# Autodesk Inventor assembly: Air Filter Bracket
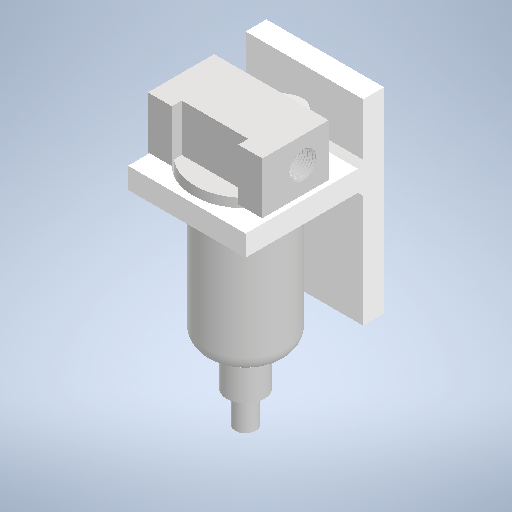
[picture p0: Inventor's stored thumbnail of the model, 512x512]
Saved by Autodesk Inventor 2025 (Build 290162000, 162)
## iProperties
Created: 2025-08-21
Part Number: Air Filter Bracket
Document SubType Name: Assembly
Designer: Caleb Fangmeier
Author: Caleb Fangmeier
## Documents named in this file (3)
- C:\Users\cfang\Desktop\nebraska-silicon-lab\Hardware\General Gantry\Air Filter Bracket\Air Filter Bracket.iam
- C:\Users\cfang\Desktop\nebraska-silicon-lab\Hardware\General Gantry\Air Filter Bracket\4274K91_Compressed Air Filter for Particle Removal\4274K91_Compressed Air Filter for Particle Removal.ipt
- C:\Users\cfang\Desktop\nebraska-silicon-lab\Hardware\General Gantry\Air Filter Bracket\Air Filter Bracket.ipt
## Components (2 placed, 2 different names)
1. 4274K91_Compressed Air Filter for Particle Removal:1 — Insert:1
2. Air Filter Bracket:1 — Insert:1
## Relationships (1: Insert 1)
- Insert:1: 4274K91_Compressed Air Filter for Particle Removal:1 ↔ Air Filter Bracket:1
